# Autodesk Inventor assembly: Brodyv2
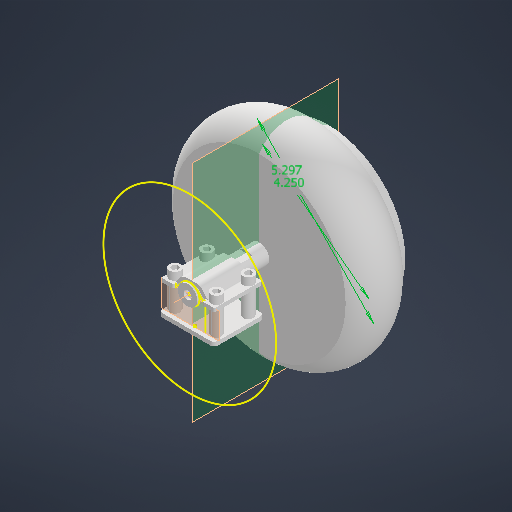
[picture p0: Inventor's stored thumbnail of the model, 512x512]
Saved by Autodesk Inventor 2027 (Build 310192000, 192)
## iProperties
Created: 2026-07-06
Part Number: Brodyv2
Document SubType Name: Assembly
Designer: belcz
Author: belcz
## Documents named in this file (6)
- C:\BrodyProject\Brodyv2.iam
- C:\BrodyProject\Wheel.ipt
- C:\BrodyProject\Wheel Bracket.ipt
- C:\BrodyProject\WheelBracketScrew.ipt
- C:\BrodyProject\WheelBracketConnector.ipt
- C:\BrodyProject\FastenerForLegFrame.ipt
## Components (8 placed, 5 different names)
1. Wheel:1 — Flush:1, Flush:2
2. Wheel Bracket:1
3. WheelBracketScrew:1
4. WheelBracketScrew:2
5. WheelBracketScrew:3
6. WheelBracketScrew:4
7. WheelBracketConnector:1
8. FastenerForLegFrame:1 — Flush:2
## Relationships (2: Flush 2)
- Flush:1 (203.2 mm): Wheel:1
- Flush:2: Wheel:1 ↔ FastenerForLegFrame:1
